# Autodesk Inventor assembly: ToughBoxMiniWith2CimMotors_MIR
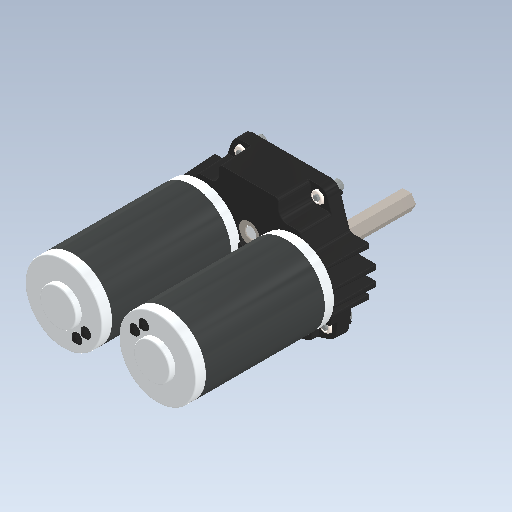
[picture p0: Inventor's stored thumbnail of the model, 512x512]
Saved by Autodesk Inventor 2020.2 (Build 242310000, 310)
## iProperties
Created: 2020-01-26
Part Number: ToughBoxMiniWith2CimMotors_MIR
Document SubType Name: Assembly
Designer: robst
Author: robst
## Documents named in this file (3)
- C:\git\CAD-Development\robSteele\2020CompetitionRobot\ToughBoxMiniWith2CimMotors_MIR.iam
- C:\git\CAD-Development\robSteele\2020CompetitionRobot\am-2598_107 2016 KOP Toughbox Mini_MIR.iam
- C:\git\CAD-Development\robSteele\2020CompetitionRobot\CIM Motor SW_MIR.ipt
## Components (3 placed, 2 different names)
1. am-2598_107 2016 KOP Toughbox Mini_MIR:1 [sub-assembly] — Insert:2, Insert:1, Insert:4, Insert:3
2. CIM Motor SW_MIR:1 — Insert:2, Insert:1
3. CIM Motor SW_MIR:2 — Insert:4, Insert:3
## Relationships (4: Insert 4)
- Insert:2: am-2598_107 2016 KOP Toughbox Mini_MIR:1 ↔ CIM Motor SW_MIR:1
- Insert:1: am-2598_107 2016 KOP Toughbox Mini_MIR:1 ↔ CIM Motor SW_MIR:1
- Insert:4: am-2598_107 2016 KOP Toughbox Mini_MIR:1 ↔ CIM Motor SW_MIR:2
- Insert:3: am-2598_107 2016 KOP Toughbox Mini_MIR:1 ↔ CIM Motor SW_MIR:2
